# Autodesk Inventor assembly: keypad
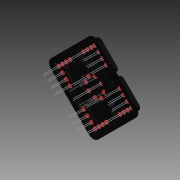
[picture p0: Inventor's stored thumbnail of the model, 180x180]
Saved by Autodesk Inventor 2015 (Build 190159000, 159)
## iProperties
Created: 2015-03-19
Part Number: keypad
Document SubType Name: Assembly
Designer: david_000
Author: david_000
## Documents named in this file (4)
- C:\Users\david_000\Dropbox\minibot\mechanics\keypad.iam
- C:\Users\david_000\Dropbox\minibot\mechanics\keypad.ipt
- C:\Users\david_000\Dropbox\minibot\mechanics\LED 5mm Red height 1-20mm\LED Heigth mm 20.0.ipt
- C:\Users\david_000\Dropbox\minibot\mechanics\LED 5mm Red height 1-20mm.ipt
## Components (37 placed, 2 different names)
1. keypad:1 — Coincidencia:1, Coincidencia:2, Coincidencia:3, Coincidencia:4, Coincidencia:5, Coincidencia:6, Coincidencia:7, Coincidencia:8, Coincidencia:9
2. LED Heigth mm 20.0:7 — Nivelación:1, Coincidencia:8
3. LED Heigth mm 20.0:6 — Nivelación:3, Coincidencia:7
4. LED Heigth mm 20.0:5 — Nivelación:2, Nivelación:3, Nivelación:4, Coincidencia:6, Nivelación:7
5. LED Heigth mm 20.0:3 — Nivelación:5, Coincidencia:5
6. LED Heigth mm 20.0:1 — Nivelación:4, Nivelación:5, Nivelación:6, Coincidencia:4
7. LED Heigth mm 20.0:2 — Nivelación:6, Coincidencia:3
8. LED Heigth mm 20.0:4 — Nivelación:1, Nivelación:2, Coincidencia:1, Coincidencia:2
9. LED Heigth mm 20.0:8
10. LED Heigth mm 20.0:9
11. LED Heigth mm 20.0:10
12. LED Heigth mm 20.0:11
13. LED Heigth mm 20.0:12
14. LED Heigth mm 20.0:13
15. LED Heigth mm 20.0:14
16. LED Heigth mm 20.0:15
17. LED Heigth mm 20.0:16
18. LED Heigth mm 20.0:17
19. LED Heigth mm 20.0:18
20. LED Heigth mm 20.0:19
21. LED Heigth mm 20.0:20
22. LED Heigth mm 20.0:21
23. LED Heigth mm 20.0:22
24. LED Heigth mm 20.0:23
25. LED Heigth mm 20.0:24
26. LED Heigth mm 20.0:25
27. LED Heigth mm 20.0:26
28. LED Heigth mm 20.0:27
29. LED Heigth mm 20.0:28
30. LED Heigth mm 20.0:29 — Coincidencia:9, Nivelación:7
31. LED Heigth mm 20.0:30
32. LED Heigth mm 20.0:31
33. LED Heigth mm 20.0:32
34. LED Heigth mm 20.0:33
35. LED Heigth mm 20.0:34
36. LED Heigth mm 20.0:35
37. LED Heigth mm 20.0:36
## Component patterns: (4 elements, first: LED Heigth mm 20.0:7 + LED Heigth mm 20.0:6 + LED Heigth mm 20.0:5 + LED Heigth mm 20.0:3 + LED Heigth mm 20.0:1 + LED Heigth mm 20.0:2 + LED Heigth mm 20.0:4), (8 elements, first: LED Heigth mm 20.0:29)
## Relationships (16: Mate 9, Flush 7)
- Nivelación:1 [Flush]: LED Heigth mm 20.0:7 ↔ LED Heigth mm 20.0:4
- Nivelación:2 [Flush]: LED Heigth mm 20.0:5 ↔ LED Heigth mm 20.0:4
- Nivelación:3 [Flush]: LED Heigth mm 20.0:6 ↔ LED Heigth mm 20.0:5
- Nivelación:4 [Flush]: LED Heigth mm 20.0:5 ↔ LED Heigth mm 20.0:1
- Nivelación:5 [Flush]: LED Heigth mm 20.0:3 ↔ LED Heigth mm 20.0:1
- Nivelación:6 [Flush]: LED Heigth mm 20.0:1 ↔ LED Heigth mm 20.0:2
- Coincidencia:1 [Mate]: keypad:1 ↔ LED Heigth mm 20.0:4
- Coincidencia:2 [Mate]: keypad:1 ↔ LED Heigth mm 20.0:4
- Coincidencia:3 [Mate]: keypad:1 ↔ LED Heigth mm 20.0:2
- Coincidencia:4 [Mate]: keypad:1 ↔ LED Heigth mm 20.0:1
- Coincidencia:5 [Mate]: keypad:1 ↔ LED Heigth mm 20.0:3
- Coincidencia:6 [Mate]: keypad:1 ↔ LED Heigth mm 20.0:5
- Coincidencia:7 [Mate]: keypad:1 ↔ LED Heigth mm 20.0:6
- Coincidencia:8 [Mate]: keypad:1 ↔ LED Heigth mm 20.0:7
- Coincidencia:9 [Mate]: keypad:1 ↔ LED Heigth mm 20.0:29
- Nivelación:7 [Flush]: LED Heigth mm 20.0:5 ↔ LED Heigth mm 20.0:29
